# Autodesk Inventor assembly: Dewalt Gear Drill Assy
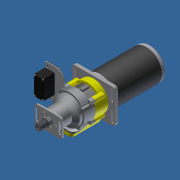
[picture p0: Inventor's stored thumbnail of the model, 180x180]
Saved by Autodesk Inventor 2012 (Build 160160000, 160)
## iProperties
Created: 2012-07-04
Part Number: Dewalt Gear Drill Assy
Document SubType Name: Assembly
Designer: Bruce
Author: Bruce
## Documents named in this file (11)
- C:\Users\Team-2471\Dropbox\Rebound Rumble 2012\Independant Swerves\Imported Components\Dewalt Gear Drill Assy.iam
- C:\Users\Team-2471\Dropbox\Rebound Rumble 2012\Independant Swerves\Imported Components\Drill Mtl Housing Dewalt XRP.ipt
- C:\Users\Team-2471\Dropbox\Rebound Rumble 2012\Independant Swerves\Imported Components\Dewalt Drill Shaft Bearing 1in x ..625 x 375.ipt
- C:\Users\Team-2471\Dropbox\Rebound Rumble 2012\Independant Swerves\Imported Components\Shaft Dewalt Drill Shaft .5in.ipt
- C:\Users\Team-2471\Dropbox\Rebound Rumble 2012\Independant Swerves\Imported Components\Drill Plastic Clamshell Housing.ipt
- C:\Users\Team-2471\Dropbox\Rebound Rumble 2012\Independant Swerves\Imported Components\Drill Motor Shifter Cover.ipt
- C:\Users\Team-2471\Dropbox\Rebound Rumble 2012\Independant Swerves\Imported Components\CIM Motor.iam
- C:\Users\Team-2471\Dropbox\Rebound Rumble 2012\Independant Swerves\Imported Components\Dewalt Drill Drive Servo Shift Mount Plate.ipt
- C:\Users\Team-2471\Dropbox\Rebound Rumble 2012\Independant Swerves\Imported Components\Hitec Servo.iam
- C:\Users\Team-2471\Dropbox\Rebound Rumble 2012\Independant Swerves\Inventor 2012\Dewalt Drill Drive CIMmotor Adaptor rectangle.ipt
- C:\Users\Team-2471\Dropbox\Rebound Rumble 2012\Independant Swerves\Inventor 2012\dewalt tom mounting plate.ipt
## Components (10 placed, 10 different names)
1. Drill Mtl Housing Dewalt XRP:1 — Mate:1, Flush:1, Flush:2, Mate:3, Mate:4, Mate:5, Mate:7, Mate:14, Mate:15, Mate:16, Mate:20, Mate:21, Mate:22
2. Dewalt Drill Shaft Bearing 1in x ..625 x 375:1 — Mate:1, Flush:1, Mate:2
3. Shaft Dewalt Drill Shaft .5in:1 — Mate:2, Flush:2
4. Drill Plastic Clamshell Housing:1 — Mate:3, Mate:4, Mate:5, Mate:6, Mate:8, Mate:9, Mate:10
5. Drill Motor Shifter Cover:1 — Mate:6, Mate:7
6. Dewalt Drill Drive CIMmotor Adaptor rectangle:1 — Mate:8, Mate:9, Mate:10, Mate:11, Mate:12, Mate:13
7. CIM Motor:1 [sub-assembly] — Mate:11, Mate:12, Mate:13
8. Dewalt Drill Drive Servo Shift Mount Plate:1 — Mate:14, Mate:15, Mate:16, Mate:17, Mate:18, Mate:19
9. Hitec Servo:1 [sub-assembly] — Mate:17, Mate:18, Mate:19
10. dewalt tom mounting plate:1 — Mate:20, Mate:21, Mate:22
## Relationships (24: Mate 22, Flush 2)
- Mate:1: Drill Mtl Housing Dewalt XRP:1 ↔ Dewalt Drill Shaft Bearing 1in x ..625 x 375:1
- Flush:1: Drill Mtl Housing Dewalt XRP:1 ↔ Dewalt Drill Shaft Bearing 1in x ..625 x 375:1
- Mate:2: Dewalt Drill Shaft Bearing 1in x ..625 x 375:1 ↔ Shaft Dewalt Drill Shaft .5in:1
- Flush:2 (-8.636 mm): Drill Mtl Housing Dewalt XRP:1 ↔ Shaft Dewalt Drill Shaft .5in:1
- Mate:3: Drill Mtl Housing Dewalt XRP:1 ↔ Drill Plastic Clamshell Housing:1
- Mate:4: Drill Mtl Housing Dewalt XRP:1 ↔ Drill Plastic Clamshell Housing:1
- Mate:5: Drill Mtl Housing Dewalt XRP:1 ↔ Drill Plastic Clamshell Housing:1
- Mate:6: Drill Plastic Clamshell Housing:1 ↔ Drill Motor Shifter Cover:1
- Mate:7 (1.016 mm): Drill Mtl Housing Dewalt XRP:1 ↔ Drill Motor Shifter Cover:1
- Mate:8: Drill Plastic Clamshell Housing:1 ↔ Dewalt Drill Drive CIMmotor Adaptor rectangle:1
- Mate:9 (0.127 mm): Drill Plastic Clamshell Housing:1 ↔ Dewalt Drill Drive CIMmotor Adaptor rectangle:1
- Mate:10: Drill Plastic Clamshell Housing:1 ↔ Dewalt Drill Drive CIMmotor Adaptor rectangle:1
- Mate:11: Dewalt Drill Drive CIMmotor Adaptor rectangle:1 ↔ CIM Motor:1
- Mate:12: Dewalt Drill Drive CIMmotor Adaptor rectangle:1 ↔ CIM Motor:1
- Mate:13: Dewalt Drill Drive CIMmotor Adaptor rectangle:1 ↔ CIM Motor:1
- Mate:14: Drill Mtl Housing Dewalt XRP:1 ↔ Dewalt Drill Drive Servo Shift Mount Plate:1
- Mate:15: Drill Mtl Housing Dewalt XRP:1 ↔ Dewalt Drill Drive Servo Shift Mount Plate:1
- Mate:16 (0.127 mm): Drill Mtl Housing Dewalt XRP:1 ↔ Dewalt Drill Drive Servo Shift Mount Plate:1
- Mate:17: Dewalt Drill Drive Servo Shift Mount Plate:1 ↔ Hitec Servo:1
- Mate:18: Dewalt Drill Drive Servo Shift Mount Plate:1 ↔ Hitec Servo:1
- Mate:19: Dewalt Drill Drive Servo Shift Mount Plate:1 ↔ Hitec Servo:1
- Mate:20: Drill Mtl Housing Dewalt XRP:1 ↔ dewalt tom mounting plate:1
- Mate:21: Drill Mtl Housing Dewalt XRP:1 ↔ dewalt tom mounting plate:1
- Mate:22: Drill Mtl Housing Dewalt XRP:1 ↔ dewalt tom mounting plate:1
